# Autodesk Inventor assembly: drivetrain
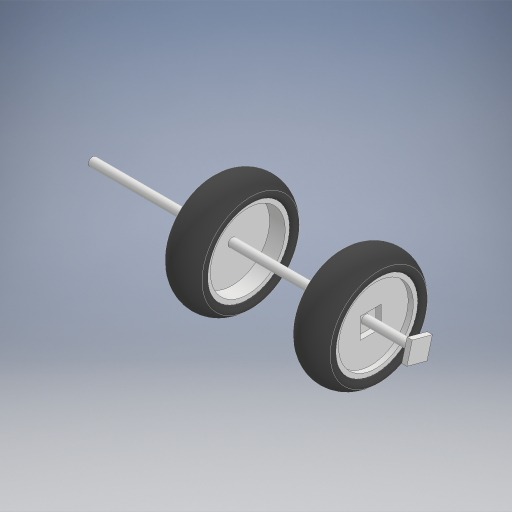
[picture p0: Inventor's stored thumbnail of the model, 512x512]
Saved by Autodesk Inventor 2024 (Build 280153000, 153)
## iProperties
Created: 2024-04-12
Part Number: drivetrain
Document SubType Name: Assembly
Designer: Alex
Author: Alex
## Documents named in this file (3)
- C:\Shared\alex-bartella-schoolwork\4z03\final\final\drivetrain.iam
- C:\Shared\alex-bartella-schoolwork\4z03\final\final\wheel.iam
- C:\Shared\alex-bartella-schoolwork\4z03\final\rear axle.ipt
## Components (3 placed, 2 different names)
1. wheel:1 [sub-assembly] — Mate:1, Mate:2
2. wheel:2 [sub-assembly] — Mate:1
3. rear axle:1 — Mate:2
## Relationships (2: Mate 2)
- Mate:1: wheel:1 ↔ wheel:2
- Mate:2: wheel:1 ↔ rear axle:1
